# Autodesk Inventor assembly: FlangedWaveguide
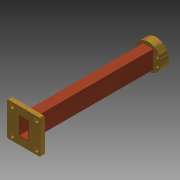
[picture p0: Inventor's stored thumbnail of the model, 180x180]
Saved by Autodesk Inventor 2015 SP1 (Build 190203100, 203)
## iProperties
Created: 2014-05-20
Part Number: FlangedWaveguide
Document SubType Name: Assembly
Designer: jad211
Author: jad211
## Documents named in this file (4)
- C:\ColdMatter\CADFiles\EDM Machine\Pumping Region\Pumping Region\FlangedWaveguide.iam
- C:\ColdMatter\CADFiles\EDM Machine\Pumping Region\Pumping Region\WG18FLANGECutDown.ipt
- C:\ColdMatter\CADFiles\EDM Machine\Pumping Region\Pumping Region\WG18 waveguide.ipt
- C:\ColdMatter\CADFiles\EDM Machine\Pumping Region\Pumping Region\WG18FLANGE.ipt
## Components (3 placed, 3 different names)
1. WG18FLANGECutDown:1 — Mate:1, Mate:2
2. WG18 waveguide:1 — Mate:1, Mate:2, Mate:3, Mate:4
3. WG18FLANGE:1 — Mate:3, Mate:4
## Relationships (4: Mate 4)
- Mate:1: WG18FLANGECutDown:1 ↔ WG18 waveguide:1
- Mate:2: WG18FLANGECutDown:1 ↔ WG18 waveguide:1
- Mate:3: WG18 waveguide:1 ↔ WG18FLANGE:1
- Mate:4: WG18 waveguide:1 ↔ WG18FLANGE:1
